# Autodesk Inventor assembly: SMALLUTM
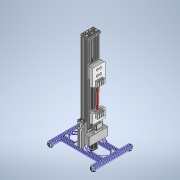
[picture p0: Inventor's stored thumbnail of the model, 180x180]
Saved by Autodesk Inventor 2022 (Build 260153000, 153)
## iProperties
Created: 2021-11-02
Part Number: SMALLUTM
Document SubType Name: Assembly
Designer: JK
Author: JK
## Documents named in this file (12)
- C:\Users\JK\Documents\Inventor\UTM\Small-Universal-Testing-Machine\CADfiles\SMALLUTM.iam
- C:\Users\JK\Documents\Inventor\UTM\Small-Universal-Testing-Machine\CADfiles\LoadCell.ipt
- C:\Users\JK\Documents\Inventor\UTM\Small-Universal-Testing-Machine\CADfiles\TensileTestSpecimen.ipt
- C:\Users\JK\Documents\Inventor\UTM\Small-Universal-Testing-Machine\CADfiles\AluminiumCouple.ipt
- C:\Users\JK\Documents\Inventor\UTM\Small-Universal-Testing-Machine\CADfiles\NEMA17.iam
- C:\Users\JK\Documents\Inventor\UTM\Small-Universal-Testing-Machine\CADfiles\GearBox.iam
- C:\Users\JK\Documents\Inventor\UTM\Small-Universal-Testing-Machine\CADfiles\Base.iam
- C:\Users\JK\Documents\Inventor\UTM\Small-Universal-Testing-Machine\CADfiles\LoadCellSupport.iam
- C:\Users\JK\Documents\Inventor\UTM\Small-Universal-Testing-Machine\CADfiles\LinearActuator.iam
- C:\Users\JK\Documents\Inventor\UTM\Small-Universal-Testing-Machine\CADfiles\UpperJawAssembly.iam
- C:\Users\JK\Documents\Inventor\UTM\Small-Universal-Testing-Machine\CADfiles\004033A Perfil aluminio (V-slot) 40×40x250.ipt
- C:\Users\JK\Documents\Inventor\UTM\Small-Universal-Testing-Machine\CADfiles\LowerJawAssembly.iam
## Components (11 placed, 11 different names)
1. LoadCell:1 — Coincidencia:111, Coincidencia:112, Ángulo:8, Coincidencia:113
2. TensileTestSpecimen:1
3. AluminiumCouple:1 — Coincidencia:81, Coincidencia:82
4. NEMA17:1 [sub-assembly] — Coincidencia:77, Coincidencia:78, Ángulo:6
5. GearBox:1 [sub-assembly] — Coincidencia:77, Coincidencia:78, Coincidencia:81, Coincidencia:82, Ángulo:6
6. Base:1 [sub-assembly] — Coincidencia:110, Nivelación:56
7. LoadCellSupport:1 [sub-assembly]
8. LinearActuator:1 [sub-assembly]
9. UpperJawAssembly:1 [sub-assembly]
10. 004033A Perfil aluminio (V-slot) 40×40x250:1 — Coincidencia:110, Nivelación:56, Coincidencia:111
11. LowerJawAssembly:1 [sub-assembly] — Coincidencia:112, Ángulo:8, Coincidencia:113
## Relationships (30: Mate 21, Flush 5, Angle 4)
- [Mate]: LoadCellSupport:1 ↔ LinearActuator:1
- [Mate]: LoadCell:1 ↔ LoadCellSupport:1
- [Angle] (0 deg): LoadCell:1 ↔ LoadCellSupport:1
- [Mate]: LoadCell:1 ↔ LoadCellSupport:1
- [Mate]: LinearActuator:1 ↔ UpperJawAssembly:1
- [Mate]: LinearActuator:1 ↔ UpperJawAssembly:1
- [Mate]: LinearActuator:1 ↔ UpperJawAssembly:1
- [Mate]: Base:1 ↔ LinearActuator:1
- [Flush]: Base:1 ↔ LinearActuator:1
- [Mate]: LoadCellSupport:1 ↔ LinearActuator:1
- [Flush]: Base:1 ↔ LoadCellSupport:1
- Coincidencia:77 [Mate]: NEMA17:1 ↔ GearBox:1
- Coincidencia:78 [Mate]: NEMA17:1 ↔ GearBox:1
- [Mate]: AluminiumCouple:1 ↔ LinearActuator:1
- [Mate]: GearBox:1 ↔ LinearActuator:1
- Coincidencia:81 [Mate] (5 mm): AluminiumCouple:1 ↔ GearBox:1
- Coincidencia:82 [Mate]: AluminiumCouple:1 ↔ GearBox:1
- [Mate]: GearBox:1 ↔ LinearActuator:1
- [Mate] (1 mm): AluminiumCouple:1 ↔ LinearActuator:1
- Ángulo:6 [Angle] (0 deg): NEMA17:1 ↔ GearBox:1
- [Angle] (180 deg): GearBox:1 ↔ Base:1
- [Flush]: NEMA17:1 ↔ Base:1
- [Mate]: Base:1 ↔ LinearActuator:1
- [Flush]: Base:1 ↔ LinearActuator:1
- Coincidencia:110 [Mate]: Base:1 ↔ 004033A Perfil aluminio (V-slot) 40×40x250:1
- Nivelación:56 [Flush]: Base:1 ↔ 004033A Perfil aluminio (V-slot) 40×40x250:1
- Coincidencia:111 [Mate]: LoadCell:1 ↔ 004033A Perfil aluminio (V-slot) 40×40x250:1
- Coincidencia:112 [Mate]: LoadCell:1 ↔ LowerJawAssembly:1
- Ángulo:8 [Angle] (0 deg): LoadCell:1 ↔ LowerJawAssembly:1
- Coincidencia:113 [Mate]: LoadCell:1 ↔ LowerJawAssembly:1
